# Autodesk Inventor assembly: top_roller
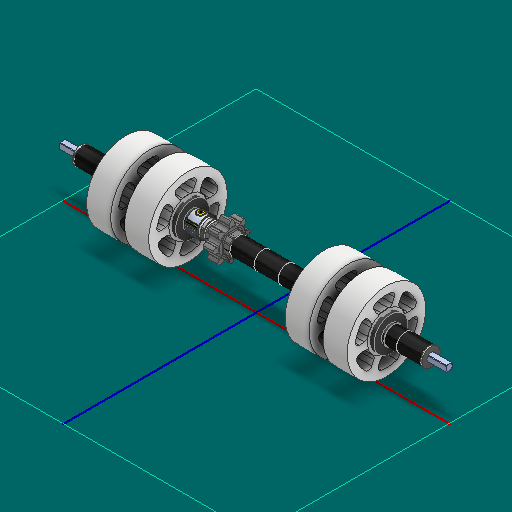
[picture p0: Inventor's stored thumbnail of the model, 512x512]
Saved by Autodesk Inventor 2025 (Build 290162000, 162)
## iProperties
Created: 2024-08-18
Part Number: top_roller
Document SubType Name: Assembly
Designer: averey
Author: averey
## Documents named in this file (18)
- C:\Users\avere\vex_robotics_high_stakes\hardware\cad\ATLAS\intake\first_stage\top_roller.iam
- C:\Users\avere\vex_robotics_high_stakes\hardware\cad\_quick_assemblies\0.8125_flex_wheel_w_versahex.iam
- C:\Users\avere\vex_robotics_high_stakes\hardware\cad\VEX-CAD-Inventor\Motion\Shaft LS\Shaft Collar ipts\Shaft Collar Set Screw.ipt
- C:\Users\avere\vex_robotics_high_stakes\hardware\cad\VEX-CAD-Inventor\Motion\Spacers\Spacer Nylon .375 OD\NSpacer .375 OD x .500.ipt
- C:\Users\avere\vex_robotics_high_stakes\hardware\cad\VEX-CAD-Inventor\Motion\Spacers\Spacer Nylon .375 OD.ipt
- C:\Users\avere\vex_robotics_high_stakes\hardware\cad\VEX-CAD-Inventor\Motion\Spacers\Spacer Nylon .375 OD\NSpacer .375 OD x .375.ipt
- C:\Users\avere\vex_robotics_high_stakes\hardware\cad\VEX-CAD-Inventor\Motion\Spacers\Washer Teflon\TWasher .375 OD x .04000.ipt
- C:\Users\avere\vex_robotics_high_stakes\hardware\cad\VEX-CAD-Inventor\Motion\Spacers\Washer Teflon.ipt
- C:\Users\avere\vex_robotics_high_stakes\hardware\cad\VEX-CAD-Inventor\Motion\Spacers\Washer Steel\SWasher .375 OD x .015625.ipt
- C:\Users\avere\vex_robotics_high_stakes\hardware\cad\VEX-CAD-Inventor\Motion\Spacers\Washer Steel.ipt
- C:\Users\avere\vex_robotics_high_stakes\hardware\cad\VEX-CAD-Inventor\Motion\Spacers\Spacer Nylon .375 OD\NSpacer .375 OD x .250.ipt
- C:\Users\avere\vex_robotics_high_stakes\hardware\cad\VEX-CAD-Inventor\Motion\Spacers\Washer Steel\SWasher .375 OD x .031250.ipt
- C:\Users\avere\vex_robotics_high_stakes\hardware\cad\VEX-CAD-Inventor\Motion\Spacers\Washer Steel\SWasher .375 OD x .062500.ipt
- C:\Users\avere\vex_robotics_high_stakes\hardware\cad\VEX-CAD-Inventor\Motion\Shaft LS\Shaft LS.ipt
- C:\Users\avere\vex_robotics_high_stakes\hardware\cad\VEX-CAD-Inventor\Motion\Shaft LS\Shaft LS\Shaft LS 8.0.ipt
- C:\Users\avere\vex_robotics_high_stakes\hardware\cad\_quick_assemblies\1.625_flex_wheel_w_versahex.iam
- C:\Users\avere\vex_robotics_high_stakes\hardware\cad\VEX-CAD-Inventor\Motion\Sprockets\6P Sprocket\6P 8T Sprocket, Circle.iam
- C:\Users\avere\vex_robotics_high_stakes\hardware\cad\VEX-CAD-Inventor\Motion\Sprockets\6P Sprocket.iam
## Components (26 placed, 12 different names)
1. 0.8125_flex_wheel_w_versahex:1 [sub-assembly] — Insert:17
2. 0.8125_flex_wheel_w_versahex:2 [sub-assembly] — Insert:25
3. 0.8125_flex_wheel_w_versahex:3 [sub-assembly] — Insert:23
4. 0.8125_flex_wheel_w_versahex:4 [sub-assembly] — Insert:14, Insert:22
5. Shaft Collar Set Screw:1
6. Shaft Collar Set Screw:2 — Insert:20, Insert:24
7. NSpacer .375 OD x .500:1
8. NSpacer .375 OD x .500:2 — Insert:26
9. NSpacer .375 OD x .500:3
10. NSpacer .375 OD x .375:4
11. TWasher .375 OD x .04000:1
12. SWasher .375 OD x .015625:1 — Insert:19
13. NSpacer .375 OD x .250:5 — Insert:13, Insert:14
14. NSpacer .375 OD x .500:6 — Insert:12, Insert:13
15. SWasher .375 OD x .031250:2 — Insert:12, Insert:21
16. NSpacer .375 OD x .250:7 — Insert:17
17. NSpacer .375 OD x .500:8
18. SWasher .375 OD x .031250:3
19. SWasher .375 OD x .062500:4 — Insert:19
20. TWasher .375 OD x .04000:2 — Insert:20
21. Shaft LS 8.0:1 — Insert:21
22. 1.625_flex_wheel_w_versahex:1 [sub-assembly] — Insert:22
23. 1.625_flex_wheel_w_versahex:2 [sub-assembly] — Insert:23
24. 1.625_flex_wheel_w_versahex:3 [sub-assembly] — Insert:24
25. 1.625_flex_wheel_w_versahex:4 [sub-assembly] — Insert:25
26. 6P 8T Sprocket, Circle:1 [sub-assembly] — Insert:26
## Relationships (26: Insert 25, Mate 1)
- [Insert]: 0.8125_flex_wheel_w_versahex:1 ↔ 0.8125_flex_wheel_w_versahex:2
- [Mate]: 0.8125_flex_wheel_w_versahex:2 ↔ 0.8125_flex_wheel_w_versahex:3
- [Insert]: 0.8125_flex_wheel_w_versahex:3 ↔ 0.8125_flex_wheel_w_versahex:4
- [Insert]: TWasher .375 OD x .04000:1 ↔ SWasher .375 OD x .015625:1
- [Insert]: NSpacer .375 OD x .500:2 ↔ TWasher .375 OD x .04000:1
- [Insert]: NSpacer .375 OD x .500:1 ↔ NSpacer .375 OD x .375:4
- [Insert]: NSpacer .375 OD x .500:1 ↔ NSpacer .375 OD x .500:3
- [Insert]: NSpacer .375 OD x .500:2 ↔ NSpacer .375 OD x .500:3
- [Insert]: 0.8125_flex_wheel_w_versahex:2 ↔ Shaft Collar Set Screw:2
- [Insert]: Shaft Collar Set Screw:1 ↔ NSpacer .375 OD x .375:4
- [Insert] (0.0424 mm): 0.8125_flex_wheel_w_versahex:3 ↔ Shaft Collar Set Screw:1
- Insert:12: NSpacer .375 OD x .500:6 ↔ SWasher .375 OD x .031250:2
- Insert:13: NSpacer .375 OD x .250:5 ↔ NSpacer .375 OD x .500:6
- Insert:14: 0.8125_flex_wheel_w_versahex:4 ↔ NSpacer .375 OD x .250:5
- [Insert]: NSpacer .375 OD x .500:8 ↔ SWasher .375 OD x .031250:3
- [Insert]: NSpacer .375 OD x .250:7 ↔ NSpacer .375 OD x .500:8
- Insert:17: 0.8125_flex_wheel_w_versahex:1 ↔ NSpacer .375 OD x .250:7
- [Insert]: SWasher .375 OD x .062500:4 ↔ TWasher .375 OD x .04000:2
- Insert:19: SWasher .375 OD x .015625:1 ↔ SWasher .375 OD x .062500:4
- Insert:20: Shaft Collar Set Screw:2 ↔ TWasher .375 OD x .04000:2
- Insert:21 (-9.525 mm): SWasher .375 OD x .031250:2 ↔ Shaft LS 8.0:1
- Insert:22: 0.8125_flex_wheel_w_versahex:4 ↔ 1.625_flex_wheel_w_versahex:1
- Insert:23: 0.8125_flex_wheel_w_versahex:3 ↔ 1.625_flex_wheel_w_versahex:2
- Insert:24: Shaft Collar Set Screw:2 ↔ 1.625_flex_wheel_w_versahex:3
- Insert:25: 0.8125_flex_wheel_w_versahex:2 ↔ 1.625_flex_wheel_w_versahex:4
- Insert:26: NSpacer .375 OD x .500:2 ↔ 6P 8T Sprocket, Circle:1
## Named parameters: d0_d9 = 0 mm, d1_d10 = 0 mm, d16_d13 = 0 mm, d17_d14 = 0 mm
